# Autodesk Inventor assembly: Frame
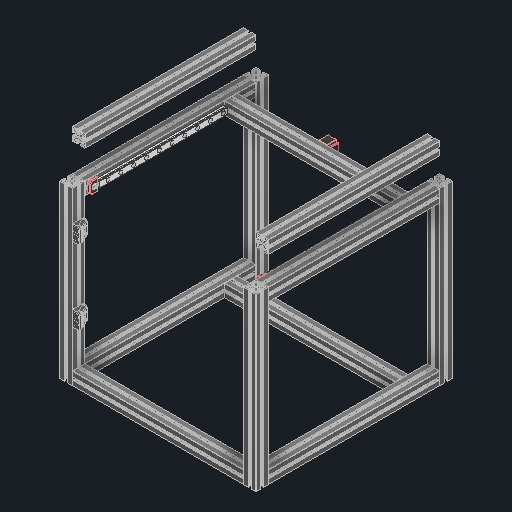
[picture p0: Inventor's stored thumbnail of the model, 512x512]
Saved by Autodesk Inventor 2025.1 (Build 291241020, 241B)
## iProperties
Created: 2025-05-09
Part Number: Frame
Document SubType Name: Assembly
Designer: AdminForWorker
Title: Frame
Author: AdminForWorker
## Documents named in this file (8)
- C:\Users\Joshua Eah\Documents\Voron 0.2\CAD\Master Assembly\Frame\Frame.iam
- C:\Users\Joshua Eah\Documents\Voron 0.2\CAD\Master Assembly\Frame\Subassemblies\Extrusions.iam
- Extrusions.iam
- C:\Users\Joshua Eah\Documents\Voron 0.2\CAD\Master Assembly\Cable Tie Assembly.iam
- C:\Users\Joshua Eah\Documents\Voron 0.2\CAD\Master Assembly\Linear Rail\MGN7 Rail 150mm.iam
- MGN7 150mm Rail.iam
- C:\Users\Joshua Eah\Documents\Voron 0.2\CAD\Master Assembly\Frame\Door Latch Assembly.iam
- C:\Users\Joshua Eah\Documents\Voron 0.2\CAD\Master Assembly\Frame\Subassemblies\Rail Stop.iam
## Components (8 placed, 5 different names)
1. Extrusions:1 [sub-assembly] — Mate:13, Mate:14, Flush:10, Flush:11, Mate:15, Mate:16, Mate:17, Flush:12, Mate:18, Mate:19, Flush:13, Mate:21, Flush:14
2. Cable Tie Assembly:1 [sub-assembly]
3. MGN7 150mm Rail:3 [sub-assembly] — Mate:13, Mate:14, Flush:10, Mate:20
4. MGN7 150mm Rail:4 [sub-assembly] — Flush:11, Mate:15, Mate:16, Mate:22
5. Door Latch Assembly:1 [sub-assembly]
6. Door Latch Assembly:2 [sub-assembly] — Mate:17, Flush:12, Mate:18
7. Rail Stop:1 [sub-assembly] — Mate:19, Mate:20, Flush:13
8. Rail Stop:2 [sub-assembly] — Mate:21, Mate:22, Flush:14
## Relationships (15: Mate 10, Flush 5)
- Mate:13: Extrusions:1 ↔ MGN7 150mm Rail:3
- Mate:14 (0.1 mm): Extrusions:1 ↔ MGN7 150mm Rail:3
- Flush:10 (38 mm): Extrusions:1 ↔ MGN7 150mm Rail:3
- Flush:11 (38 mm): Extrusions:1 ↔ MGN7 150mm Rail:4
- Mate:15: Extrusions:1 ↔ MGN7 150mm Rail:4
- Mate:16 (0.1 mm): Extrusions:1 ↔ MGN7 150mm Rail:4
- Mate:17: Extrusions:1 ↔ Door Latch Assembly:2
- Flush:12: Extrusions:1 ↔ Door Latch Assembly:2
- Mate:18 (44.54 mm): Extrusions:1 ↔ Door Latch Assembly:2
- Mate:19: Extrusions:1 ↔ Rail Stop:1
- Mate:20: MGN7 150mm Rail:3 ↔ Rail Stop:1
- Flush:13: Extrusions:1 ↔ Rail Stop:1
- Mate:21: Extrusions:1 ↔ Rail Stop:2
- Mate:22: MGN7 150mm Rail:4 ↔ Rail Stop:2
- Flush:14: Extrusions:1 ↔ Rail Stop:2
